# Autodesk Inventor assembly: 01hand
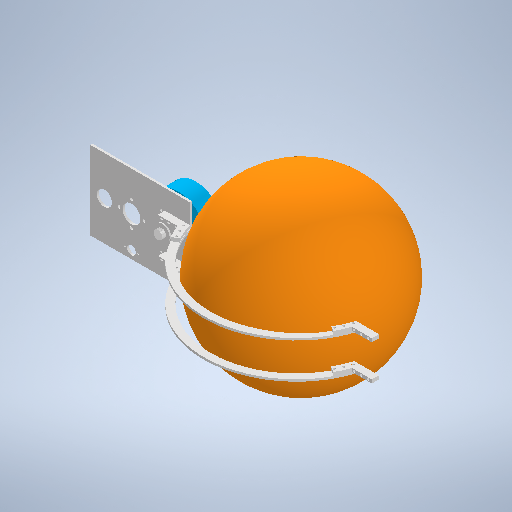
[picture p0: Inventor's stored thumbnail of the model, 512x512]
Saved by Autodesk Inventor 2025.1 (Build 291241000, 241)
## iProperties
Created: 2025-05-01
Part Number: 01hand
Document SubType Name: Assembly
Designer: yuki0520
Author: yuki0520
## Documents named in this file (9)
- C:\Users\yuki0520\OneDrive\ドキュメント\Inventor\2025_nhk\tanaka\drible\01hand.iam
- C:\Users\yuki0520\OneDrive\ドキュメント\Inventor\2025_nhk\tanaka\drible\ring_to_plate.ipt
- C:\Users\yuki0520\OneDrive\ドキュメント\Inventor\2025_nhk\tanaka\drible\ring.ipt
- C:\Users\yuki0520\OneDrive\ドキュメント\Inventor\2025_nhk\tanaka\drible\dr_plate_motor.ipt
- C:\Users\yuki0520\OneDrive\ドキュメント\Inventor\2025_nhk\tanaka\nageru\smallring\small_bar_roller.ipt
- C:\Users\yuki0520\OneDrive\ドキュメント\Inventor\2025_nhk\tanaka\nageru\pakuriz\bear_12_18.ipt
- C:\Users\yuki0520\OneDrive\ドキュメント\Inventor\2025_nhk\tanaka\nageru\smallring\small_tire.ipt
- C:\Users\yuki0520\OneDrive\ドキュメント\Inventor\2025_nhk\tanaka\nageru\smallring\small_tire_fixer.ipt
- C:\Users\yuki0520\OneDrive\ドキュメント\Inventor\2025_nhk\tanaka\object\ball.ipt
## Components (13 placed, 8 different names)
1. ring_to_plate:1 — 挿入:1, 挿入:4
2. ring_to_plate:2 — 挿入:2, 挿入:3, 挿入:9, 挿入:10
3. ring:1 — 挿入:1, 挿入:2, 挿入:3, 挿入:4
4. ring_to_plate:3
5. ring_to_plate:4 — 挿入:11, 挿入:12
6. ring:2
7. dr_plate_motor:1 — 挿入:9, 挿入:10, 挿入:11, 挿入:12, メイト:1, メイト:2, フラッシュ:1
8. small_bar_roller:1 — メイト:3, メイト:4, メイト:5, メイト:6, フラッシュ:1
9. bear_12_18:1 — メイト:1, メイト:2, メイト:3
10. small_tire:1 — 挿入:13, 挿入:14, 挿入:15, 挿入:16, 正接:1
11. small_tire_fixer:1 — 挿入:15, 挿入:16, メイト:6
12. small_tire_fixer:2 — 挿入:13, 挿入:14, メイト:4, メイト:5
13. ball:1 — 正接:1
## Relationships (24: Insert 16, Mate 6, Flush 1, Tangent 1)
- 挿入:1 [Insert]: ring_to_plate:1 ↔ ring:1
- 挿入:2 [Insert]: ring_to_plate:2 ↔ ring:1
- 挿入:3 [Insert]: ring_to_plate:2 ↔ ring:1
- 挿入:4 [Insert]: ring_to_plate:1 ↔ ring:1
- [Insert]: ring_to_plate:3 ↔ ring:2
- [Insert]: ring_to_plate:4 ↔ ring:2
- [Insert]: ring_to_plate:4 ↔ ring:2
- [Insert]: ring_to_plate:3 ↔ ring:2
- 挿入:9 [Insert]: ring_to_plate:2 ↔ dr_plate_motor:1
- 挿入:10 [Insert]: ring_to_plate:2 ↔ dr_plate_motor:1
- 挿入:11 [Insert]: ring_to_plate:4 ↔ dr_plate_motor:1
- 挿入:12 [Insert]: ring_to_plate:4 ↔ dr_plate_motor:1
- メイト:1 [Mate]: dr_plate_motor:1 ↔ bear_12_18:1
- メイト:2 [Mate]: dr_plate_motor:1 ↔ bear_12_18:1
- メイト:3 [Mate]: small_bar_roller:1 ↔ bear_12_18:1
- 挿入:13 [Insert]: small_tire:1 ↔ small_tire_fixer:2
- 挿入:14 [Insert]: small_tire:1 ↔ small_tire_fixer:2
- 挿入:15 [Insert]: small_tire:1 ↔ small_tire_fixer:1
- 挿入:16 [Insert]: small_tire:1 ↔ small_tire_fixer:1
- メイト:4 [Mate]: small_bar_roller:1 ↔ small_tire_fixer:2
- メイト:5 [Mate]: small_bar_roller:1 ↔ small_tire_fixer:2
- メイト:6 [Mate]: small_bar_roller:1 ↔ small_tire_fixer:1
- フラッシュ:1 [Flush] (7 mm): dr_plate_motor:1 ↔ small_bar_roller:1
- 正接:1 [Tangent]: small_tire:1 ↔ ball:1
## Named parameters: d4_d0 = 0 mm, d5_d1 = 0 mm, d6_d2 = 0 mm, d7_d3 = 0 mm
